# Autodesk Inventor assembly: NOTGATEASSEMBLY
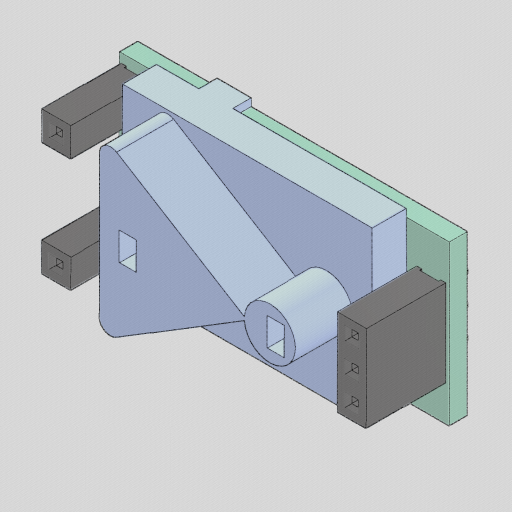
[picture p0: Inventor's stored thumbnail of the model, 512x512]
Saved by Autodesk Inventor 2024.3 (Build 283343000, 343)
## iProperties
Created: 2024-01-22
Part Number: NOTGATEASSEMBLY
Document SubType Name: Assembly
Designer: Jetsan
Author: Jetsan
## Documents named in this file (3)
- C:\Git\DigitalLogicProject\Models\NOTGATE\NOTGATEASSEMBLY.iam
- C:\Git\DigitalLogicProject\Models\ANDGATE\ANDGATE.iam
- C:\Git\DigitalLogicProject\Models\NOTGATE\NOTGATE.ipt
## Components (2 placed, 2 different names)
1. ANDGATE:1 [sub-assembly] — Mate:1, Mate:2
2. NOTGATE:1 — Mate:1, Mate:2
## Relationships (2: Mate 2)
- Mate:1: ANDGATE:1 ↔ NOTGATE:1
- Mate:2: ANDGATE:1 ↔ NOTGATE:1
